# Autodesk Inventor assembly: Montagem Amassador
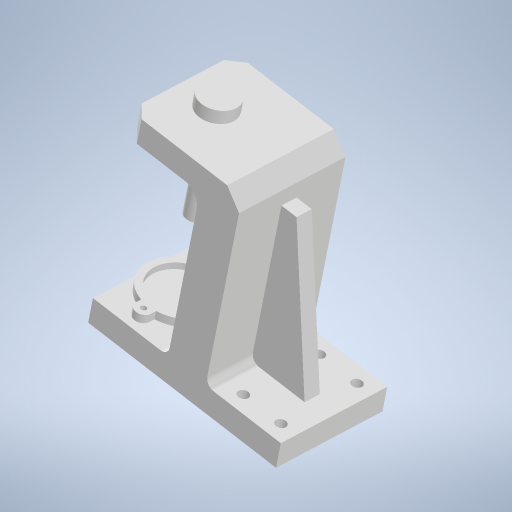
[picture p0: Inventor's stored thumbnail of the model, 512x512]
Saved by Autodesk Inventor 2023.2 (Build 272271000, 271)
## iProperties
Created: 2022-12-19
Part Number: Montagem Amassador
Document SubType Name: Assembly
Designer: coqui
Author: coqui
## Documents named in this file (4)
- D:\Felipe Coquito\OneDrive\Documents\Inventor\Inventor - curso\Montagem\Montagem Amassador.iam
- D:\Felipe Coquito\OneDrive\Documents\Inventor\Inventor - curso\Amassador\Base do Amassador.ipt
- D:\Felipe Coquito\OneDrive\Documents\Inventor\Inventor - curso\Amassador\Prato do Amassador.ipt
- D:\Felipe Coquito\OneDrive\Documents\Inventor\Inventor - curso\Amassador\Pino do Amassador.ipt
## Components (3 placed, 3 different names)
1. Base do Amassador:1 — Mate:1, Mate:2, Mate:3, Angle:1, Mate:4, Mate:5
2. Prato do Amassador:1 — Mate:1, Mate:2, Mate:3
3. Pino do Amassador:1 — Angle:1, Mate:4, Mate:5
## Relationships (6: Mate 5, Angle 1)
- Mate:1: Base do Amassador:1 ↔ Prato do Amassador:1
- Mate:2: Base do Amassador:1 ↔ Prato do Amassador:1
- Mate:3: Base do Amassador:1 ↔ Prato do Amassador:1
- Angle:1 (0 deg): Base do Amassador:1 ↔ Pino do Amassador:1
- Mate:4: Base do Amassador:1 ↔ Pino do Amassador:1
- Mate:5: Base do Amassador:1 ↔ Pino do Amassador:1
